# Autodesk Inventor assembly: voltage_regulator_with_pins
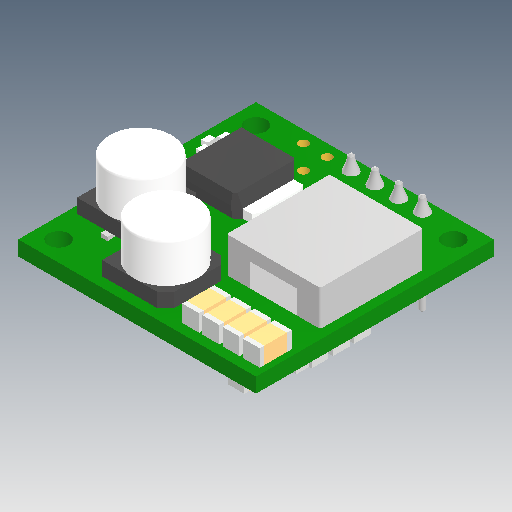
[picture p0: Inventor's stored thumbnail of the model, 512x512]
Saved by Autodesk Inventor 2020 (Build 240168000, 168)
## iProperties
Created: 2020-09-27
Part Number: voltage_regulator_with_pins
Document SubType Name: Assembly
Designer: DELL
Author: DELL
## Documents named in this file (3)
- F:\SoftRobot\Model\FlexipodHardware-master\mechanical_model\5V_5.5A_Voltage_Regulator_D36V50F5\voltage_regulator_with_pins.iam
- F:\SoftRobot\Model\FlexipodHardware-master\mechanical_model\5V_5.5A_Voltage_Regulator_D36V50F5\step_down_voltage_regulator.ipt
- F:\SoftRobot\Model\FlexipodHardware-master\mechanical_model\pins.ipt
## Components (5 placed, 2 different names)
1. step_down_voltage_regulator:1 — Mate:1, Mate:2, Angle:1
2. pins:1 — Mate:1, Mate:2, Angle:1
3. pins:2
4. pins:3
5. pins:4
## Component patterns: (4 elements, first: pins:1)
## Relationships (3: Mate 2, Angle 1)
- Mate:1: step_down_voltage_regulator:1 ↔ pins:1
- Mate:2: step_down_voltage_regulator:1 ↔ pins:1
- Angle:1 (0 deg): step_down_voltage_regulator:1 ↔ pins:1
